# Autodesk Inventor assembly: motorizedSwitchHanger
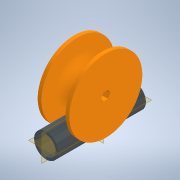
[picture p0: Inventor's stored thumbnail of the model, 180x180]
Saved by Autodesk Inventor 2020.2 (Build 242310000, 310)
## iProperties
Created: 2020-01-06
Part Number: motorizedSwitchHanger
Document SubType Name: Assembly
Designer: steele
Author: steele
## Documents named in this file (3)
- C:\git\CAD-Development\robSteele\2020 Lift Mechanism\motorizedSwitchHanger.iam
- C:\git\CAD-Development\robSteele\2020 Lift Mechanism\switchHangingPipe.ipt
- C:\git\CAD-Development\robSteele\2020 Lift Mechanism\wheelForHangingAndMoving.ipt
## Components (2 placed, 2 different names)
1. switchHangingPipe:1 — Flush:1, Flush:2, Flush:3
2. wheelForHangingAndMoving:1 — Flush:1, Flush:2, Flush:3
## Relationships (3: Flush 3)
- Flush:1: switchHangingPipe:1 ↔ wheelForHangingAndMoving:1
- Flush:2: switchHangingPipe:1 ↔ wheelForHangingAndMoving:1
- Flush:3 (50.8 mm): switchHangingPipe:1 ↔ wheelForHangingAndMoving:1
